# Autodesk Inventor assembly: Assembly
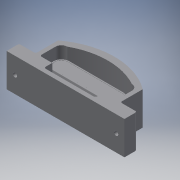
[picture p0: Inventor's stored thumbnail of the model, 180x180]
Saved by Autodesk Inventor 2017 (Build 210142000, 142)
## iProperties
Part Number: Assembly
Material: 一般
Document SubType Name: Assembly
Designer: taige
Author: taige
## Documents named in this file (3)
- C:\Users\taige\Documents\Inventor\RealSense\Assembly.iam
- C:\Users\taige\Documents\Inventor\RealSense\jig.ipt
- C:\Users\taige\Desktop\Intel_RealSense_Depth_Camera_D435.STEP_\Intel_RealSense_Depth_Camera_D435.iam
## Components (2 placed, 2 different names)
1. jig:1 — メイト:1, メイト:2, メイト:3
2. Intel_RealSense_Depth_Camera_D435:1 [sub-assembly] — メイト:1, メイト:2, メイト:3
## Relationships (3: Mate 3)
- メイト:1 [Mate]: jig:1 ↔ Intel_RealSense_Depth_Camera_D435:1
- メイト:2 [Mate]: jig:1 ↔ Intel_RealSense_Depth_Camera_D435:1
- メイト:3 [Mate]: jig:1 ↔ Intel_RealSense_Depth_Camera_D435:1
